# Autodesk Inventor assembly: disassembled
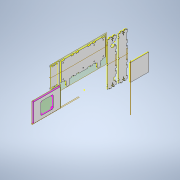
[picture p0: Inventor's stored thumbnail of the model, 180x180]
Saved by Autodesk Inventor 2020 (Build 240168000, 168)
## iProperties
Created: 2020-01-09
Part Number: disassembled
Document SubType Name: Assembly
Designer: erwin
Author: erwin
## Documents named in this file (8)
- D:\GitHub\ElCheapoAIS-nmea\case\Wooden Multicase\prototype\disassembled.iam
- D:\GitHub\ElCheapoAIS-nmea\case\Wooden Multicase\prototype\side_side.ipt
- D:\GitHub\ElCheapoAIS-nmea\case\Wooden Multicase\prototype\cover_wires.ipt
- D:\GitHub\ElCheapoAIS-nmea\case\Wooden Multicase\prototype\cover_components.ipt
- D:\GitHub\ElCheapoAIS-nmea\case\Wooden Multicase\prototype\cover.ipt
- D:\GitHub\ElCheapoAIS-nmea\case\Wooden Multicase\prototype\drawings_easel.ipt
- D:\GitHub\ElCheapoAIS-nmea\case\Wooden Multicase\prototype\new_side_top.ipt
- D:\GitHub\ElCheapoAIS-nmea\case\Wooden Multicase\prototype\new_side_bottom.ipt
## Components (7 placed, 7 different names)
1. cover:1 — Flush:3, Flush:4, Flush:9
2. cover_components:1 — Flush:5, Flush:7, Flush:8
3. cover_wires:1 — Flush:10
4. side_side:2
5. new_side_top:1 — Flush:3, Flush:5
6. new_side_bottom:1 — Flush:4, Flush:10
7. drawings_easel:1 — Flush:7, Flush:8, Flush:9
## Relationships (7: Flush 7)
- Flush:3: cover:1 ↔ new_side_top:1
- Flush:4: cover:1 ↔ new_side_bottom:1
- Flush:5: cover_components:1 ↔ new_side_top:1
- Flush:7: cover_components:1 ↔ drawings_easel:1
- Flush:8: cover_components:1 ↔ drawings_easel:1
- Flush:9: cover:1 ↔ drawings_easel:1
- Flush:10: cover_wires:1 ↔ new_side_bottom:1
